# Autodesk Inventor assembly: Remote
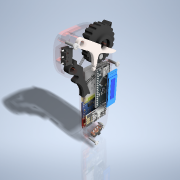
[picture p0: Inventor's stored thumbnail of the model, 180x180]
Saved by Autodesk Inventor 2020.1 (Build 241239000, 239)
## iProperties
Created: 2019-07-16
Part Number: Remote
Document SubType Name: Assembly
Designer: Petar
Author: Petar
## Documents named in this file (25)
- D:\OMG\E-Board\CAD\Inventor\Remote\Remote.iam
- D:\OMG\E-Board\CAD\Inventor\Remote\Remote Top Shell.ipt
- D:\OMG\E-Board\CAD\Inventor\Remote\Trigger.ipt
- D:\OMG\E-Board\CAD\Inventor\Remote\Remote Bottom Shell.ipt
- D:\OMG\E-Board\CAD\Inventor\Electrical Components\Cirquit Parts\Microswitch Subminiature Lever SPDT Through Hole.ipt
- D:\OMG\E-Board\CAD\Inventor\Electrical Components\Cirquit Parts\Slide Switch\SPDT Mini Slide Switch.iam
- D:\OMG\E-Board\CAD\Inventor\Electrical Components\LiPo 502535.ipt
- D:\OMG\E-Board\CAD\Inventor\Electrical Components\TP4056 Board\Lipo Charger - TP4056.iam
- D:\OMG\E-Board\CAD\Inventor\Electrical Components\LED Screen 0.91 inch.ipt
- D:\OMG\E-Board\CAD\Inventor\Electrical Components\Arduino Nano\arduino nano.iam
- D:\OMG\E-Board\CAD\Inventor\Electrical Components\DC-DC RT9266.ipt
- D:\OMG\E-Board\CAD\Inventor\Electrical Components\Cirquit Parts\Halleffect Sensor SS495A1.ipt
- D:\OMG\E-Board\CAD\Inventor\Electrical Components\Magnets 5x5.ipt
- D:\OMG\E-Board\CAD\Inventor\Electrical Components\Cirquit Parts\micro_usb_47346-0001.ipt
- D:\OMG\E-Board\CAD\Inventor\Remote\Springy.ipt
- D:\OMG\E-Board\CAD\Inventor\Remote\Plate.ipt
- D:\OMG\E-Board\CAD\Inventor\Electrical Components\nRF24L01+_enhanced.ipt
- D:\OMG\E-Board\CAD\Inventor\Other\Acrylic Plate.ipt
- D:\OMG\E-Board\CAD\Inventor\Remote\Remote\Design Accelerator\Bolted Connection1.iam
- D:\OMG\E-Board\CAD\Inventor\Remote\Remote\Design Accelerator\Bolted Connection2.iam
- D:\OMG\E-Board\CAD\Inventor\Remote\Remote\Design Accelerator\Bolted Connection3.iam
- D:\OMG\E-Board\CAD\Inventor\Remote\Spring.ipt
- D:\OMG\E-Board\CAD\Inventor\Remote\Knob_v2.ipt
- D:\OMG\E-Board\CAD\Inventor\Remote\Spring 2.ipt
- D:\OMG\E-Board\CAD\Inventor\Electrical Components\LED WS2812B.ipt
## Components (25 placed, 22 different names)
1. Remote Top Shell:1 — Rigid:14, Rigid:19, Rigid:24, Mate:1, Mate:3, Mate:5
2. Remote Bottom Shell:1 — Rigid:2, Rotational:1, Rotational:2, Rigid:8, Rigid:10, Rigid:13, Rigid:14, Rotational:3, Rigid:18, Rigid:20, Rigid:23, Mate:2, Mate:4, Mate:6, Mate:8
3. Knob_v2:1 — Rigid:3, Rigid:4, Rotational:1
4. Trigger:1 — Rotational:2
5. Plate:1 — Rigid:20, Rigid:21, Rigid:22, Rigid:25
6. LED WS2812B:1
7. Microswitch Subminiature Lever SPDT Through Hole:1 — Rigid:23
8. Spring:1 — Mate:7, Mate:8
9. SPDT Mini Slide Switch:1 [sub-assembly] — Rigid:8
10. LiPo 502535:1 — Rigid:13
11. Lipo Charger - TP4056:1 [sub-assembly] — Rigid:10, Rigid:16
12. DC-DC RT9266:1 — Rigid:16
13. Halleffect Sensor SS495A1:1 — Rigid:2
14. Magnets 5x5:1 — Rigid:4
15. Magnets 5x5:2 — Rigid:3
16. micro_usb_47346-0001:1 — Rigid:18
17. Springy:1 — Rotational:3, Mate:7
18. Spring 2:1 — Rigid:25
19. Acrylic Plate:1 — Rigid:24
20. nRF24L01+_enhanced:1 — Rigid:22
21. LED Screen 0.91 inch:1 — Rigid:19
22. arduino nano:1 [sub-assembly] — Rigid:21
23. Bolted Connection:1 [sub-assembly] — Mate:1, Mate:2
24. Bolted Connection:2 [sub-assembly] — Mate:3, Mate:4
25. Bolted Connection:3 [sub-assembly] — Mate:5, Mate:6
## Relationships (27: WeldJoint 16, Mate 8, RevoluteJoint 3)
- Rigid:2 [WeldJoint]: Remote Bottom Shell:1 ↔ Halleffect Sensor SS495A1:1
- Rigid:3 [WeldJoint]: Knob_v2:1 ↔ Magnets 5x5:2
- Rigid:4 [WeldJoint]: Knob_v2:1 ↔ Magnets 5x5:1
- Rotational:1 [RevoluteJoint] (0.2 mm): Remote Bottom Shell:1 ↔ Knob_v2:1
- Rotational:2 [RevoluteJoint]: Remote Bottom Shell:1 ↔ Trigger:1
- Rigid:8 [WeldJoint]: Remote Bottom Shell:1 ↔ SPDT Mini Slide Switch:1
- Rigid:10 [WeldJoint]: Remote Bottom Shell:1 ↔ Lipo Charger - TP4056:1
- Rigid:13 [WeldJoint]: Remote Bottom Shell:1 ↔ LiPo 502535:1
- Rigid:14 [WeldJoint]: Remote Top Shell:1 ↔ Remote Bottom Shell:1
- Rigid:16 [WeldJoint]: Lipo Charger - TP4056:1 ↔ DC-DC RT9266:1
- Rotational:3 [RevoluteJoint]: Remote Bottom Shell:1 ↔ Springy:1
- Rigid:18 [WeldJoint]: Remote Bottom Shell:1 ↔ micro_usb_47346-0001:1
- Rigid:19 [WeldJoint]: Remote Top Shell:1 ↔ LED Screen 0.91 inch:1
- Rigid:20 [WeldJoint]: Remote Bottom Shell:1 ↔ Plate:1
- Rigid:21 [WeldJoint]: Plate:1 ↔ arduino nano:1
- Rigid:22 [WeldJoint]: Plate:1 ↔ nRF24L01+_enhanced:1
- Rigid:23 [WeldJoint]: Remote Bottom Shell:1 ↔ Microswitch Subminiature Lever SPDT Through Hole:1
- Rigid:24 [WeldJoint]: Remote Top Shell:1 ↔ Acrylic Plate:1
- Mate:1: Remote Top Shell:1 ↔ Bolted Connection:1
- Mate:2: Remote Bottom Shell:1 ↔ Bolted Connection:1
- Mate:3: Remote Top Shell:1 ↔ Bolted Connection:2
- Mate:4: Remote Bottom Shell:1 ↔ Bolted Connection:2
- Mate:5: Remote Top Shell:1 ↔ Bolted Connection:3
- Mate:6: Remote Bottom Shell:1 ↔ Bolted Connection:3
- Mate:7: Spring:1 ↔ Springy:1
- Mate:8: Remote Bottom Shell:1 ↔ Spring:1
- Rigid:25 [WeldJoint] (-0.15 mm): Plate:1 ↔ Spring 2:1
